# Autodesk Inventor assembly: Ensamblaje1
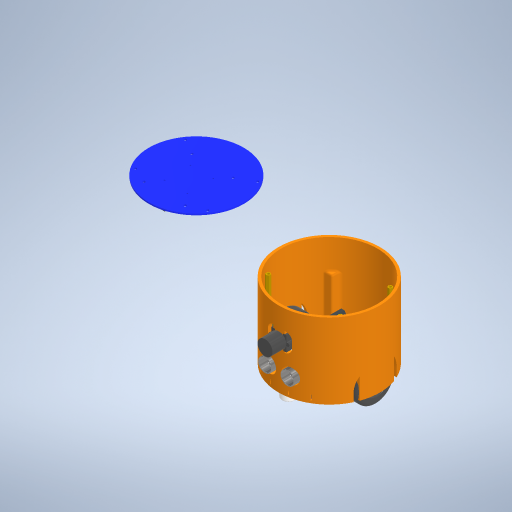
[picture p0: Inventor's stored thumbnail of the model, 512x512]
Saved by Autodesk Inventor 2023 (Build 270158000, 158)
## iProperties
Created: 2022-07-23
Part Number: Ensamblaje1
Document SubType Name: Assembly
Designer: LJNC
Author: LJNC
## Documents named in this file (7)
- C:\Users\LJNC\Desktop\Alphabot\Ensamblaje1.iam
- C:\Users\LJNC\Desktop\Alphabot\Inferior.ipt
- C:\Users\LJNC\Desktop\Alphabot\Carcaza.ipt
- C:\Users\LJNC\Desktop\Alphabot\Espaciador_40mm.ipt
- C:\Users\LJNC\Desktop\Alphabot\Alphabot_SUP.ipt
- C:\Users\LJNC\Desktop\Alphabot\US.ipt
- C:\Users\LJNC\Desktop\Alphabot\PiCam.ipt
## Components (11 placed, 6 different names)
1. Inferior:1 — Rígido:1
2. Carcaza:1 — Rígido:1, Rígido:4, Rígido:6, Rígido:8, Rígido:9, Rígido:10
3. Espaciador_40mm:1 — Rígido:2, Rígido:4
4. Espaciador_40mm:2 — Rígido:2
5. Espaciador_40mm:3 — Rígido:8
6. Espaciador_40mm:4
7. Espaciador_40mm:5 — Rígido:6
8. Espaciador_40mm:6 — Rígido:7
9. Alphabot_SUP:1 — Rígido:7
10. US:1 — Rígido:9
11. PiCam:1 — Rígido:10
## Relationships (10: WeldJoint 10)
- Rígido:1 [WeldJoint]: Inferior:1 ↔ Carcaza:1
- Rígido:2 [WeldJoint]: Espaciador_40mm:1 ↔ Espaciador_40mm:2
- [WeldJoint]: Espaciador_40mm:3 ↔ Espaciador_40mm:4
- Rígido:4 [WeldJoint]: Carcaza:1 ↔ Espaciador_40mm:1
- [WeldJoint]: Espaciador_40mm:5 ↔ Espaciador_40mm:6
- Rígido:6 [WeldJoint]: Carcaza:1 ↔ Espaciador_40mm:5
- Rígido:7 [WeldJoint]: Espaciador_40mm:6 ↔ Alphabot_SUP:1
- Rígido:8 [WeldJoint]: Carcaza:1 ↔ Espaciador_40mm:3
- Rígido:9 [WeldJoint]: Carcaza:1 ↔ US:1
- Rígido:10 [WeldJoint] (2.5 mm): Carcaza:1 ↔ PiCam:1
## Named parameters: d4_d3 = 0 mm, d6_d4_d3 = 0 mm
